# Autodesk Inventor assembly: Дверка45
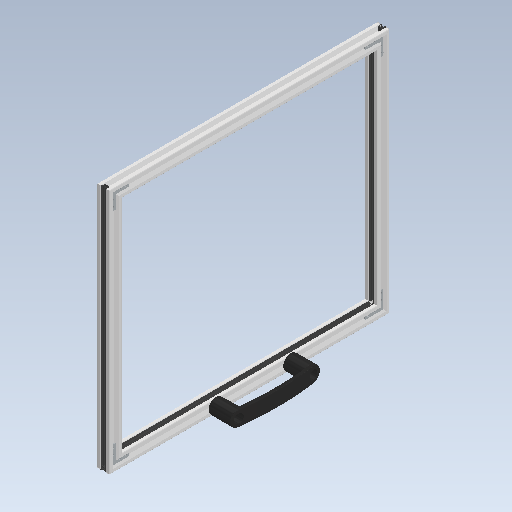
[picture p0: Inventor's stored thumbnail of the model, 512x512]
Saved by Autodesk Inventor 2020 (Build 240168000, 168)
## iProperties
Created: 2020-04-04
Part Number: Дверка45
Document SubType Name: Assembly
Designer: Михаил
Author: Михаил
## Documents named in this file (9)
- D:\MyWorks\GrowBox_v2\Box\3D_body\Дверка45.iam
- D:\MyWorks\GrowBox_v2\Box\3D_body\Профиль_аллюминиевый395_45.ipt
- D:\MyWorks\GrowBox_v2\Box\3D_body\Профиль_аллюминиевый450_45.ipt
- D:\MyWorks\GrowBox_v2\Box\3D_body\Vnutrenniy-soedinitel-20-seriya.T15.ipt
- D:\MyWorks\GrowBox_v2\Box\3D_body\Ruchka-dvernaya-plastikovaya_-120mm_T10_.ipt
- D:\MyWorks\GrowBox_v2\Box\3D_body\Uplotnitel-pazovyy355_-paz-6.ipt
- D:\MyWorks\GrowBox_v2\Box\3D_body\Uplotnitel-pazovyy410_-paz-6.ipt
- D:\MyWorks\GrowBox_v2\Box\3D_body\Uplotnitel-pazovyy450_-paz-6.ipt
- D:\MyWorks\GrowBox_v2\Box\3D_body\Uplotnitel-pazovyy395_-paz-6.ipt
## Components (16 placed, 7 different names)
1. Профиль_алюминиевый:1 — Совмещение:1, Заподлицо:1, Угол:1, Заподлицо:2, Совмещение:2, Заподлицо:3, Совмещение:5, Совмещение:7, Совмещение:8, Совмещение:15, Совмещение:18, Заподлицо:5, Совмещение:21
2. Профиль_алюминиевый:2 — Совмещение:1, Заподлицо:1, Угол:1, Заподлицо:2, Совмещение:3, Заподлицо:4, Совмещение:6, Совмещение:10, Совмещение:12, Совмещение:14, Совмещение:20, Заподлицо:6
3. Профиль_алюминиевый:3 — Совмещение:2, Заподлицо:3, Совмещение:3, Совмещение:4, Совмещение:16, Совмещение:19, Заподлицо:7
4. Профиль_алюминиевый:4 — Совмещение:4, Заподлицо:4, Совмещение:5, Совмещение:9, Совмещение:13, Совмещение:17, Совмещение:22
5. Vnutrenniy-soedinitel-20-seriya.T15:1 — Совмещение:6
6. Vnutrenniy-soedinitel-20-seriya.T15:2 — Совмещение:7
7. Vnutrenniy-soedinitel-20-seriya.T15:3 — Совмещение:8
8. Vnutrenniy-soedinitel-20-seriya.T15:4 — Совмещение:9
9. Ruchka-dvernaya-plastikovaya_-120mm_T10_:1 — Совмещение:10
10. Uplotnitel-pazovyy355_-paz-6:1 — Совмещение:12, Совмещение:13
11. Uplotnitel-pazovyy410_-paz-6:1 — Совмещение:14, Совмещение:15
12. Uplotnitel-pazovyy355_-paz-6:2 — Совмещение:18, Совмещение:19
13. Uplotnitel-pazovyy410_-paz-6:2 — Совмещение:16, Совмещение:17
14. Uplotnitel-pazovyy450_-paz-6:1 — Совмещение:20, Заподлицо:5
15. Uplotnitel-pazovyy395_-paz-6:1 — Совмещение:22, Заподлицо:7
16. Uplotnitel-pazovyy395_-paz-6:2 — Совмещение:21, Заподлицо:6
## Relationships (29: Mate 21, Flush 7, Angle 1)
- Совмещение:1 [Mate]: Профиль_алюминиевый:1 ↔ Профиль_алюминиевый:2
- Заподлицо:1 [Flush]: Профиль_алюминиевый:1 ↔ Профиль_алюминиевый:2
- Угол:1 [Angle] (90 deg): Профиль_алюминиевый:1 ↔ Профиль_алюминиевый:2
- Заподлицо:2 [Flush]: Профиль_алюминиевый:1 ↔ Профиль_алюминиевый:2
- Совмещение:2 [Mate]: Профиль_алюминиевый:1 ↔ Профиль_алюминиевый:3
- Заподлицо:3 [Flush]: Профиль_алюминиевый:1 ↔ Профиль_алюминиевый:3
- Совмещение:3 [Mate] (355 mm): Профиль_алюминиевый:2 ↔ Профиль_алюминиевый:3
- Совмещение:4 [Mate]: Профиль_алюминиевый:3 ↔ Профиль_алюминиевый:4
- Заподлицо:4 [Flush]: Профиль_алюминиевый:2 ↔ Профиль_алюминиевый:4
- Совмещение:5 [Mate] (410 mm): Профиль_алюминиевый:1 ↔ Профиль_алюминиевый:4
- Совмещение:6 [Mate]: Профиль_алюминиевый:2 ↔ Vnutrenniy-soedinitel-20-seriya.T15:1
- Совмещение:7 [Mate]: Профиль_алюминиевый:1 ↔ Vnutrenniy-soedinitel-20-seriya.T15:2
- Совмещение:8 [Mate]: Профиль_алюминиевый:1 ↔ Vnutrenniy-soedinitel-20-seriya.T15:3
- Совмещение:9 [Mate]: Профиль_алюминиевый:4 ↔ Vnutrenniy-soedinitel-20-seriya.T15:4
- Совмещение:10 [Mate]: Профиль_алюминиевый:2 ↔ Ruchka-dvernaya-plastikovaya_-120mm_T10_:1
- Совмещение:12 [Mate]: Профиль_алюминиевый:2 ↔ Uplotnitel-pazovyy355_-paz-6:1
- Совмещение:13 [Mate]: Профиль_алюминиевый:4 ↔ Uplotnitel-pazovyy355_-paz-6:1
- Совмещение:14 [Mate]: Профиль_алюминиевый:2 ↔ Uplotnitel-pazovyy410_-paz-6:1
- Совмещение:15 [Mate]: Профиль_алюминиевый:1 ↔ Uplotnitel-pazovyy410_-paz-6:1
- Совмещение:16 [Mate]: Профиль_алюминиевый:3 ↔ Uplotnitel-pazovyy410_-paz-6:2
- Совмещение:17 [Mate]: Профиль_алюминиевый:4 ↔ Uplotnitel-pazovyy410_-paz-6:2
- Совмещение:18 [Mate]: Профиль_алюминиевый:1 ↔ Uplotnitel-pazovyy355_-paz-6:2
- Совмещение:19 [Mate]: Профиль_алюминиевый:3 ↔ Uplotnitel-pazovyy355_-paz-6:2
- Совмещение:20 [Mate]: Профиль_алюминиевый:2 ↔ Uplotnitel-pazovyy450_-paz-6:1
- Заподлицо:5 [Flush]: Профиль_алюминиевый:1 ↔ Uplotnitel-pazovyy450_-paz-6:1
- Совмещение:21 [Mate]: Профиль_алюминиевый:1 ↔ Uplotnitel-pazovyy395_-paz-6:2
- Заподлицо:6 [Flush]: Профиль_алюминиевый:2 ↔ Uplotnitel-pazovyy395_-paz-6:2
- Совмещение:22 [Mate]: Профиль_алюминиевый:4 ↔ Uplotnitel-pazovyy395_-paz-6:1
- Заподлицо:7 [Flush]: Профиль_алюминиевый:3 ↔ Uplotnitel-pazovyy395_-paz-6:1
